# Autodesk Inventor assembly: Polea Compuesta
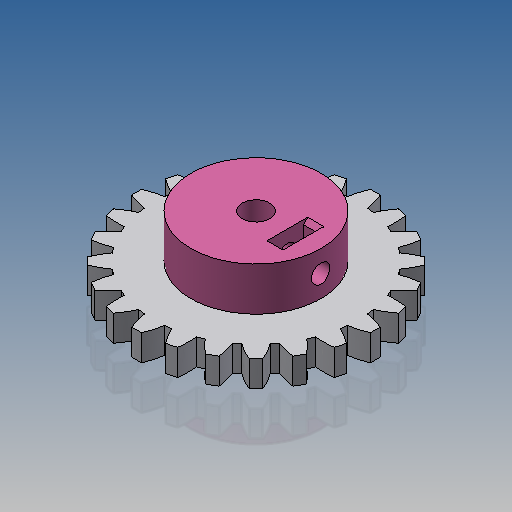
[picture p0: Inventor's stored thumbnail of the model, 512x512]
Saved by Autodesk Inventor 2017 (Build 210142000, 142)
## iProperties
Part Number: Polea Compuesta
Material: Genérico
Document SubType Name: Assembly
Designer: FABLAB
Author: FABLAB
## Documents named in this file (5)
- C:\Users\Leo\Documents\GitHub\actor-re-actor\models\inventor-caja\transmision Engranajes\Polea Compuesta.iam
- C:\Users\Leo\Documents\GitHub\actor-re-actor\models\inventor-caja\transmision Engranajes\dado polea.ipt
- C:\Users\Leo\Documents\GitHub\actor-re-actor\models\inventor-caja\transmision Engranajes\engrane motor-dado.ipt
- C:\Users\FABLAB\Documents\Inventor\Content Center Files\R2017\es-ES\AS 1112 (2)\AS 1112 - M4  Tipo 5.ipt
- C:\Users\FABLAB\Documents\Inventor\Content Center Files\R2017\es-ES\AS 1421(4)\AS 1421 - M3 x 10 Punta plana.ipt
## Components (4 placed, 4 different names)
1. dado polea:1 — Nivelación:1, Insertar:1
2. engrane motor-dado:1 — Nivelación:1, Coincidencia:1, Coincidencia:2
3. AS 1112 (2) - Métrico M4  Tipo 5:1 — Insertar:1, Coincidencia:3
4. AS 1421 Punta plana - Métrico M3 x 10 Punta plana:1 — Coincidencia:3
## Relationships (5: Mate 3, Flush 1, Insert 1)
- Nivelación:1 [Flush]: dado polea:1 ↔ engrane motor-dado:1
- Coincidencia:1 [Mate]: engrane motor-dado:1
- Coincidencia:2 [Mate]: engrane motor-dado:1
- Insertar:1: dado polea:1 ↔ AS 1112 (2) - Métrico M4  Tipo 5:1
- Coincidencia:3 [Mate]: AS 1112 (2) - Métrico M4  Tipo 5:1 ↔ AS 1421 Punta plana - Métrico M3 x 10 Punta plana:1
